# Autodesk Inventor assembly: slide assembly
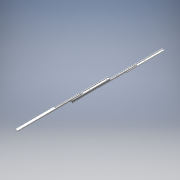
[picture p0: Inventor's stored thumbnail of the model, 180x180]
Saved by Autodesk Inventor 2019 (Build 230136000, 136)
## iProperties
Created: 2019-05-04
Part Number: slide assembly
Document SubType Name: Assembly
Designer: Delta
Author: Delta
## Documents named in this file (3)
- C:\Robotics\2019-20_CAD\offseason\random ideas\slides\slide assembly.iam
- C:\Robotics\COTSParts\Misumi_Slides\AIS2018\SAR330.iam
- C:\Robotics\2019-20_CAD\offseason\random ideas\slides\slide conector.ipt
## Components (3 placed, 2 different names)
1. SAR330:1 [sub-assembly] — Mate:1, Mate:2, Mate:3
2. SAR330:2 [sub-assembly] — Mate:4, Mate:5, Mate:6
3. slide conector:1 — Mate:1, Mate:2, Mate:3, Mate:4, Mate:5, Mate:6
## Relationships (6: Mate 6)
- Mate:1: SAR330:1 ↔ slide conector:1
- Mate:2: SAR330:1 ↔ slide conector:1
- Mate:3: SAR330:1 ↔ slide conector:1
- Mate:4: SAR330:2 ↔ slide conector:1
- Mate:5: SAR330:2 ↔ slide conector:1
- Mate:6: SAR330:2 ↔ slide conector:1
